# Autodesk Inventor assembly: ShiftRail
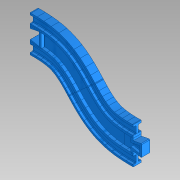
[picture p0: Inventor's stored thumbnail of the model, 180x180]
Saved by Autodesk Inventor 2021 (Build 250183000, 183)
## iProperties
Created: 2021-06-08
Part Number: ShiftRail
Document SubType Name: Assembly
Designer: kumagai
Author: kumagai
## Documents named in this file (4)
- X:\Develop\CAD\PlaRails\ShiftRail\ShiftRail.iam
- X:\Develop\CAD\PlaRails\ShiftRail\RailJointDSFemale.ipt
- X:\Develop\CAD\PlaRails\ShiftRail\RailJointDSMale.ipt
- X:\Develop\CAD\PlaRails\ShiftRail\ShiftRail_TC.ipt
## Components (4 placed, 3 different names)
1. ShiftRail_TC:1 — フラッシュ:2, フラッシュ:3, メイト:3
2. ShiftRail_TC:2 — フラッシュ:4, フラッシュ:5, メイト:4
3. RailJointDSFemale:1 — フラッシュ:4, フラッシュ:5, メイト:4
4. RailJointDSMale:1 — フラッシュ:2, フラッシュ:3, メイト:3
## Relationships (9: Flush 5, Mate 4)
- [Flush]: ShiftRail_TC:1 ↔ ShiftRail_TC:2
- [Mate]: ShiftRail_TC:1 ↔ ShiftRail_TC:2
- [Mate]: ShiftRail_TC:1 ↔ ShiftRail_TC:2
- フラッシュ:2 [Flush]: ShiftRail_TC:1 ↔ RailJointDSMale:1
- フラッシュ:3 [Flush]: ShiftRail_TC:1 ↔ RailJointDSMale:1
- メイト:3 [Mate]: ShiftRail_TC:1 ↔ RailJointDSMale:1
- フラッシュ:4 [Flush]: ShiftRail_TC:2 ↔ RailJointDSFemale:1
- フラッシュ:5 [Flush]: ShiftRail_TC:2 ↔ RailJointDSFemale:1
- メイト:4 [Mate]: ShiftRail_TC:2 ↔ RailJointDSFemale:1
